# Autodesk Inventor assembly: Clutch Assembly
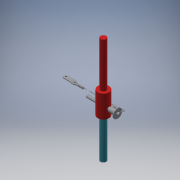
[picture p0: Inventor's stored thumbnail of the model, 180x180]
Saved by Autodesk Inventor 2016 (Build 200138000, 138)
## iProperties
Created: 2015-06-15
Part Number: Clutch Assembly
Document SubType Name: Assembly
Designer: steele
Author: steele
## Documents named in this file (4)
- C:\snobotics\CAD\robSteele\Bevel Gearbox\2015 Summer Bevel Gearbox\Clutch Assembly.iam
- C:\snobotics\CAD\robSteele\Bevel Gearbox\2015 Summer Bevel Gearbox\Part of Clutch.ipt
- C:\snobotics\CAD\robSteele\Bevel Gearbox\2015 Summer Bevel Gearbox\Lower Half of Clutch.ipt
- C:\snobotics\CAD\partResources\McMaster-Carr\quickReleasePin\94748A227.ipt
## Components (3 placed, 3 different names)
1. Part of Clutch:1 — Insert:1, Mate:1
2. Lower Half of Clutch:1 — Insert:1
3. 94748A227:1 — Mate:1
## Relationships (2: Insert 1, Mate 1)
- Insert:1: Part of Clutch:1 ↔ Lower Half of Clutch:1
- Mate:1: Part of Clutch:1 ↔ 94748A227:1
